# Autodesk Inventor assembly: ROV Control Pipe Assembly
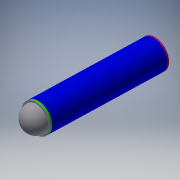
[picture p0: Inventor's stored thumbnail of the model, 180x180]
Saved by Autodesk Inventor 2016 (Build 200138000, 138)
## iProperties
Created: 2017-01-19
Part Number: ROV Control Pipe Assembly
Document SubType Name: Assembly
Designer: Student
Author: Student
## Documents named in this file (8)
- C:\Users\Student\Desktop\Noah Code\ROV Control Pipe Assembly.iam
- C:\Users\Student\Desktop\Noah Code\4 inch PVC pipe.ipt
- C:\Users\Student\Documents\Raspberry Pi.ipt
- C:\Users\Student\Documents\arduino uno.ipt
- C:\Users\Student\Desktop\O ring Plug 1.ipt
- C:\Users\Student\Desktop\O ring Dome 2.ipt
- C:\Users\Student\Desktop\Noah Code\RPI camera.ipt
- C:\Users\Student\Desktop\Noah Code\ROV Dome 4''.ipt
## Components (7 placed, 7 different names)
1. 4 inch PVC pipe:1 — Mate:1, Mate:2, Mate:3
2. Raspberry Pi:1
3. arduino uno:1
4. O ring Plug 1:1 — Mate:1
5. O ring Dome 2:1 — Mate:2, Mate:3, Mate:4
6. RPI camera:1
7. ROV Dome 4'':1 — Mate:4
## Relationships (4: Mate 4)
- Mate:1: 4 inch PVC pipe:1 ↔ O ring Plug 1:1
- Mate:2: 4 inch PVC pipe:1 ↔ O ring Dome 2:1
- Mate:3: 4 inch PVC pipe:1 ↔ O ring Dome 2:1
- Mate:4: O ring Dome 2:1 ↔ ROV Dome 4'':1
